# Autodesk Inventor assembly: T-Copter
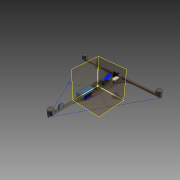
[picture p0: Inventor's stored thumbnail of the model, 180x180]
Saved by Autodesk Inventor 2012 (Build 160160000, 160)
## iProperties
Created: 2013-02-28
Part Number: T-Copter
Document SubType Name: Assembly
Designer: fixer
Mass: 785.259 g
Surface Area: 2464 cm^2
Volume: 686.799 cm^3
Density: 1.14336 g/cm^3
RuleStatus: InUse
Author: fixer
## Documents named in this file (16)
- C:\Users\fixer\Documents\Inventor\T-Copter\T-Copter.iam
- C:\Users\fixer\Documents\Inventor\T-Copter\Arm.ipt
- C:\Users\fixer\Documents\Inventor\T-Copter\Rangelink Reciever.ipt
- C:\Users\fixer\Documents\Inventor\T-Copter\Video Tx.ipt
- C:\Users\fixer\Documents\Inventor\T-Copter\Lisa-M.ipt
- C:\Users\fixer\Documents\Inventor\T-Copter\HK 20A BEC.ipt
- C:\Users\fixer\Documents\Inventor\T-Copter\Battery - 3S 2200mAh.ipt
- C:\Users\fixer\Documents\Inventor\T-Copter\Rear Arm.ipt
- C:\Users\fixer\Documents\Inventor\T-Copter\Triangle.ipt
- C:\Users\fixer\Documents\Inventor\T-Copter\Camera - SONY CCD.ipt
- C:\Users\fixer\Documents\Inventor\T-Copter\Top Plate.ipt
- C:\Users\fixer\Documents\Inventor\T-Copter\Servo.ipt
- C:\Users\fixer\Documents\Inventor\T-Copter\Front Spacer.ipt
- C:\Users\fixer\Documents\Inventor\T-Copter\Side Spacer.ipt
- C:\Users\fixer\Documents\Inventor\T-Copter\Bottom Plate v2.ipt
- C:\Users\fixer\Documents\Inventor\T-Copter\Motor - DT750.ipt
## Components (21 placed, 16 different names)
1. Rangelink Reciever — Mate:12
2. Video Tx — Mate:25, Mate:42
3. Lisa-M — Mate:11, Mate:39
4. Battery - 3S 2200mAh — Mate:24, Mate:41
5. ESC - HK 20A:1 — Mate:8
6. ESC - HK 20A:3 — Mate:10
7. HK 20A BEC:4
8. Camera - SONY CCD — Mate:26
9. Servo — Mate:27, Mate:28
10. Motor - DT750:1 — Flush:15, Flush:16, Tangent:3
11. Motor - DT750:2 — Mate:43, Mate:45, Tangent:2
12. Motor - DT750:3 — Mate:44, Mate:46, Tangent:1
13. Triangle — Mate:18, Mate:19, Mate:20, Mate:45, Mate:46
14. Bottom Plate — Flush:5, Mate:8, Mate:10, Mate:11, Mate:12, Mate:15, Flush:11, Flush:12, Mate:29, Mate:32, Mate:33, Mate:34, Mate:35, Mate:36, Mate:37, Flush:14
15. Top Plate — Flush:13, Mate:40, Flush:14, Mate:41, Mate:42
16. Side Spacer:2 — Mate:33, Mate:34, Mate:36
17. Side Spacer:1 — Mate:32, Mate:35, Mate:37
18. Front Spacer:1 — Mate:29, Mate:30, Mate:31
19. Arm — Mate:4, Flush:12, Mate:20, Mate:30, Mate:43, Tangent:2
20. Arm:2 — Mate:5, Flush:11, Mate:19, Mate:44, Tangent:1
21. Rear Arm — Mate:3, Mate:18, Mate:27, Flush:15, Tangent:3
## Relationships (44: Mate 33, Flush 8, Tangent 3)
- Mate:3: Rear Arm
- Flush:5: Bottom Plate
- Mate:4: Arm
- Mate:5: Arm:2
- Flush:6 (6.35 mm)
- Mate:8: ESC - HK 20A:1 ↔ Bottom Plate
- Mate:10: ESC - HK 20A:3 ↔ Bottom Plate
- Mate:11: Lisa-M ↔ Bottom Plate
- Mate:12: Rangelink Reciever ↔ Bottom Plate
- Mate:15 (-6.35 mm): Bottom Plate
- Flush:11: Bottom Plate ↔ Arm:2
- Flush:12: Bottom Plate ↔ Arm
- Mate:18: Triangle ↔ Rear Arm
- Mate:19: Triangle ↔ Arm:2
- Mate:20: Triangle ↔ Arm
- Mate:24: Battery - 3S 2200mAh
- Mate:25: Video Tx
- Mate:26: Camera - SONY CCD
- Mate:27: Servo ↔ Rear Arm
- Mate:28: Servo
- Mate:29: Bottom Plate ↔ Front Spacer:1
- Mate:30: Front Spacer:1 ↔ Arm
- Mate:31: Front Spacer:1
- Mate:32: Bottom Plate ↔ Side Spacer:1
- Mate:33: Bottom Plate ↔ Side Spacer:2
- Mate:34: Bottom Plate ↔ Side Spacer:2
- Mate:35: Bottom Plate ↔ Side Spacer:1
- Mate:36 (25.4 mm): Bottom Plate ↔ Side Spacer:2
- Mate:37 (25.4 mm): Bottom Plate ↔ Side Spacer:1
- Mate:39: Lisa-M
- Flush:13: Top Plate
- Mate:40: Top Plate
- Flush:14: Bottom Plate ↔ Top Plate
- Mate:41: Battery - 3S 2200mAh ↔ Top Plate
- Mate:42: Video Tx ↔ Top Plate
- Flush:15: Motor - DT750:1 ↔ Rear Arm
- Flush:16: Motor - DT750:1
- Mate:43: Motor - DT750:2 ↔ Arm
- Mate:44: Motor - DT750:3 ↔ Arm:2
- Mate:45: Motor - DT750:2 ↔ Triangle
- Mate:46: Motor - DT750:3 ↔ Triangle
- Tangent:1: Motor - DT750:3 ↔ Arm:2
- Tangent:2: Motor - DT750:2 ↔ Arm
- Tangent:3: Motor - DT750:1 ↔ Rear Arm
